# Autodesk Inventor assembly: Locking Pin Assy
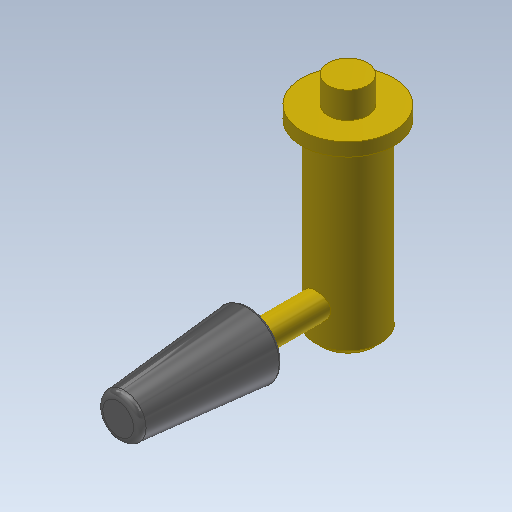
[picture p0: Inventor's stored thumbnail of the model, 512x512]
Saved by Autodesk Inventor 2020 (Build 240168000, 168)
## iProperties
Created: 2012-11-06
Part Number: Locking Pin Assy
Document SubType Name: Assembly
Designer: Lance
Mass: 0.468859 g
Surface Area: 6.68049 cm^2
Volume: 0.476775 cm^3
Density: 0.983398 g/cm^3
Author: Lance
## Documents named in this file (4)
- C:\Users\Hesekiel\Desktop\MUM\Mechanika\Mechanizm elewacji i elektronika Filip\CAD\manfrotto-494rc2-tripod-head.snapshot.1\Manfrotto 494RC2 - Tripod Head\Locking Pin Assy.iam
- C:\Users\Hesekiel\Desktop\MUM\Mechanika\Mechanizm elewacji i elektronika Filip\CAD\manfrotto-494rc2-tripod-head.snapshot.1\Manfrotto 494RC2 - Tripod Head\Locking Pin.ipt
- C:\Users\Hesekiel\Desktop\MUM\Mechanika\Mechanizm elewacji i elektronika Filip\CAD\manfrotto-494rc2-tripod-head.snapshot.1\Manfrotto 494RC2 - Tripod Head\Locking Pin Lever.ipt
- C:\Users\Hesekiel\Desktop\MUM\Mechanika\Mechanizm elewacji i elektronika Filip\CAD\manfrotto-494rc2-tripod-head.snapshot.1\Manfrotto 494RC2 - Tripod Head\Locking Pin Lever Rubber.ipt
## Components (3 placed, 3 different names)
1. Locking Pin:1 — Mate:1, Tangent:1, Flush:1
2. Locking Pin Lever:1 — Mate:1, Tangent:1, Flush:1, Insert:1, Flush:2
3. Locking Pin Lever Rubber:1 — Insert:1, Flush:2
## Relationships (5: Flush 2, Mate 1, Tangent 1, Insert 1)
- Mate:1: Locking Pin:1 ↔ Locking Pin Lever:1
- Tangent:1: Locking Pin:1 ↔ Locking Pin Lever:1
- Flush:1: Locking Pin:1 ↔ Locking Pin Lever:1
- Insert:1: Locking Pin Lever:1 ↔ Locking Pin Lever Rubber:1
- Flush:2: Locking Pin Lever:1 ↔ Locking Pin Lever Rubber:1
